# Autodesk Inventor assembly: 22205/20 E
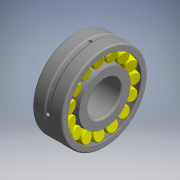
[picture p0: Inventor's stored thumbnail of the model, 180x180]
Saved by Autodesk Inventor 2017.3 (Build 213256000, 256)
## iProperties
Category: PARTsolutions
Company: SKF
Part Number: 22205/20 E
Catalog Web Link: www.cadenas.de
Description: BS2_001-Spherical roller bearings
Vendor: SKF
Document SubType Name: Assembly
Designer: partserver
Manufacturer: SKF
Mass: 280 g
Surface Area: 167.54 cm^2
Volume: 24.1426 cm^3
Density: 11.5977 g/cm^3
Title: 22205/20 E
Author: Cadenas PARTsolutions
Comments: Spherical roller bearings
PSOL_IDENT_0: {$CADENAS_DATA\23d-libs\skf\bearings_units_and_housings\roller_bearings\spherical_roller_bearings\bs
PSOL_IDENT_1: 2_001.prj},179 {VTYP=3D},{STYP=ASSTAB},{NB=22205/20 E},{LINA=22205/20 E},{NN=BS2_001},{DATE=23.12.20
PSOL_IDENT_2: 20 07:01:43},{GEOMDATE=14.12.2020 11:44:40},{VERSION=},{LINEID=460970},{WBVAR=},{WBNUMERIC=}  {NB=22
PSOL_IDENT_3: 205/20 E},{LINA=22205/20 E},{KT=DUMMY},{DESIGNATION=22205/20 E},{VARIANT=CE1W33},{DESIGNX=Cylindrica
PSOL_IDENT_4: l bore},{SEAL=No seals},{SALG=NO},{BORE=20.000},{DD=20.000},{DD1=MIN},{D=52.000},{B=18.000},{DD2=31.
PSOL_IDENT_5: 300},{DD3=MIN},{D1=44.200},{B1=MIN},{B2=MIN},{B4=MIN},{B5=MIN},{BB=3.700},{K=2.000},{R12=1.000},{G=}
PSOL_IDENT_6: ,{G1=MIN},{TB=MIN},{ALPHA=12.8333},{R34=MIN},{PITCH=39.459},{DW=7.130},{LW=6.600},{DDAMIN=25.600},{D
PSOL_IDENT_7: DAMAX=MIN},{DBMIN=MIN},{DAMAX=46.400},{BAMIN=MIN},{RAMAX=1.000},{LOAD1=49.900},{LOAD2=44.000},{LOAD3=
PSOL_IDENT_8: 4.750},{SPEED1=13000},{SPEED2=17000},{PRA=},{PLA=},{Z=15.000},{II=2.000},{MASS=0.280},{MASS2=MIN},{S
PSOL_IDENT_9: LEEVE=},{POPULAR=},{BEARING=22205/20 E},{PPATH=parts/bs2_001_asmtpl.prj},{RAMAXX=1},{EE=0.35},{Y0=1.
PSOL_IDENT_10: 8},{R12X=1},{Y2=2.9},{ALPHAX=12.83333},{Y1=1.9},{DD1X=},{B1X=},{SLEEVEX=},{ALPHAXX=},{B2X=},{SUPRESS
PSOL_IDENT_11: ED=},{BBALG=3.700},{KALG=2.000}
NB: 22205/20 E
NN: BS2_001
NT: Spherical roller bearings
NBSYN: $DESIGNATION.
LINA: 22205/20 E
CATALOG: SKF
DESIGNATION: 22205/20 E
DESIGNX: Cylindrical bore
SEAL: No seals
BORE: 20
D: 52
B: 18
LOAD1: 49.9
LOAD2: 44
LOAD3: 4.75
SPEED1: 13000
SPEED2: 17000
SUPPLIER: SKF
ARTICLENO: 22205/20 E
BOMINFO: 22205/20 E
CREATOR: CADENAS GmbH
## Documents named in this file (6)
- e:\temp\worker_18\temp\exporttempdir_6528_6_YBdq6\format_0\22205_20 E.iam
- e:\temp\worker_18\temp\exporttempdir_6528_6_YBdq6\format_0\22205_20 E_dummy.ipt
- e:\temp\worker_18\temp\exporttempdir_6528_6_YBdq6\format_0\22205_20 E_ir.ipt
- e:\temp\worker_18\temp\exporttempdir_6528_6_YBdq6\format_0\22205_20 E_or.ipt
- e:\temp\worker_18\temp\exporttempdir_6528_6_YBdq6\format_0\22205_20 E_r1.ipt
- e:\temp\worker_18\temp\exporttempdir_6528_6_YBdq6\format_0\22205_20 E_r2.ipt
## Components (33 placed, 5 different names)
1. 22205_20 E_dummy:1 — dummy_XY@1 <-> ir_XY@2, dummy_Z@1 <-> ir_Z@2, dummy_YZ@1 <-> ir_YZ@2, dummy_XY@1 <-> or_XY@3, dummy_Z@1 <-> or_Z@3, dummy_YZ@1 <-> or_YZ@3, roller1_XY@1 <-> roller1_XY@4, roller1_Z@1 <-> roller1_Z@4, roller1_YZ@1 <-> roller1_YZ@4, roller1_XY@1 <-> roller2_XY@5, roller1_Z@1 <-> roller2_Z@5, roller1_YZ@1 <-> roller2_YZ@5, roller2_XY@1 <-> roller1_XY@6, roller2_Z@1 <-> roller1_Z@6, roller2_YZ@1 <-> roller1_YZ@6, roller2_XY@1 <-> roller2_XY@7, roller2_Z@1 <-> roller2_Z@7, roller2_YZ@1 <-> roller2_YZ@7, roller3_XY@1 <-> roller1_XY@8, roller3_Z@1 <-> roller1_Z@8, roller3_YZ@1 <-> roller1_YZ@8, roller3_XY@1 <-> roller2_XY@9, roller3_Z@1 <-> roller2_Z@9, roller3_YZ@1 <-> roller2_YZ@9, roller4_XY@1 <-> roller1_XY@10, roller4_Z@1 <-> roller1_Z@10, roller4_YZ@1 <-> roller1_YZ@10, roller4_XY@1 <-> roller2_XY@11, roller4_Z@1 <-> roller2_Z@11, roller4_YZ@1 <-> roller2_YZ@11, roller5_XY@1 <-> roller1_XY@12, roller5_Z@1 <-> roller1_Z@12, roller5_YZ@1 <-> roller1_YZ@12, roller5_XY@1 <-> roller2_XY@13, roller5_Z@1 <-> roller2_Z@13, roller5_YZ@1 <-> roller2_YZ@13, roller6_XY@1 <-> roller1_XY@14, roller6_Z@1 <-> roller1_Z@14, roller6_YZ@1 <-> roller1_YZ@14, roller6_XY@1 <-> roller2_XY@15, roller6_Z@1 <-> roller2_Z@15, roller6_YZ@1 <-> roller2_YZ@15, roller7_XY@1 <-> roller1_XY@16, roller7_Z@1 <-> roller1_Z@16, roller7_YZ@1 <-> roller1_YZ@16, roller7_XY@1 <-> roller2_XY@17, roller7_Z@1 <-> roller2_Z@17, roller7_YZ@1 <-> roller2_YZ@17, roller8_XY@1 <-> roller1_XY@18, roller8_Z@1 <-> roller1_Z@18, roller8_YZ@1 <-> roller1_YZ@18, roller8_XY@1 <-> roller2_XY@19, roller8_Z@1 <-> roller2_Z@19, roller8_YZ@1 <-> roller2_YZ@19, roller9_XY@1 <-> roller1_XY@20, roller9_Z@1 <-> roller1_Z@20, roller9_YZ@1 <-> roller1_YZ@20, roller9_XY@1 <-> roller2_XY@21, roller9_Z@1 <-> roller2_Z@21, roller9_YZ@1 <-> roller2_YZ@21, roller10_XY@1 <-> roller1_XY@22, roller10_Z@1 <-> roller1_Z@22, roller10_YZ@1 <-> roller1_YZ@22, roller10_XY@1 <-> roller2_XY@23, roller10_Z@1 <-> roller2_Z@23, roller10_YZ@1 <-> roller2_YZ@23, roller11_XY@1 <-> roller1_XY@24, roller11_Z@1 <-> roller1_Z@24, roller11_YZ@1 <-> roller1_YZ@24, roller11_XY@1 <-> roller2_XY@25, roller11_Z@1 <-> roller2_Z@25, roller11_YZ@1 <-> roller2_YZ@25, roller12_XY@1 <-> roller1_XY@26, roller12_Z@1 <-> roller1_Z@26, roller12_YZ@1 <-> roller1_YZ@26, roller12_XY@1 <-> roller2_XY@27, roller12_Z@1 <-> roller2_Z@27, roller12_YZ@1 <-> roller2_YZ@27, roller13_XY@1 <-> roller1_XY@28, roller13_Z@1 <-> roller1_Z@28, roller13_YZ@1 <-> roller1_YZ@28, roller13_XY@1 <-> roller2_XY@29, roller13_Z@1 <-> roller2_Z@29, roller13_YZ@1 <-> roller2_YZ@29, roller14_XY@1 <-> roller1_XY@30, roller14_Z@1 <-> roller1_Z@30, roller14_YZ@1 <-> roller1_YZ@30, roller14_XY@1 <-> roller2_XY@31, roller14_Z@1 <-> roller2_Z@31, roller14_YZ@1 <-> roller2_YZ@31, roller15_XY@1 <-> roller1_XY@32, roller15_Z@1 <-> roller1_Z@32, roller15_YZ@1 <-> roller1_YZ@32, roller15_XY@1 <-> roller2_XY@33, roller15_Z@1 <-> roller2_Z@33, roller15_YZ@1 <-> roller2_YZ@33
2. 22205_20 E_ir:1 — dummy_XY@1 <-> ir_XY@2, dummy_Z@1 <-> ir_Z@2, dummy_YZ@1 <-> ir_YZ@2
3. 22205_20 E_or:1 — dummy_XY@1 <-> or_XY@3, dummy_Z@1 <-> or_Z@3, dummy_YZ@1 <-> or_YZ@3
4. 22205_20 E_r1:1 — roller1_XY@1 <-> roller1_XY@4, roller1_Z@1 <-> roller1_Z@4, roller1_YZ@1 <-> roller1_YZ@4
5. 22205_20 E_r2:1 — roller1_XY@1 <-> roller2_XY@5, roller1_Z@1 <-> roller2_Z@5, roller1_YZ@1 <-> roller2_YZ@5
6. 22205_20 E_r1:2 — roller2_XY@1 <-> roller1_XY@6, roller2_Z@1 <-> roller1_Z@6, roller2_YZ@1 <-> roller1_YZ@6
7. 22205_20 E_r2:2 — roller2_XY@1 <-> roller2_XY@7, roller2_Z@1 <-> roller2_Z@7, roller2_YZ@1 <-> roller2_YZ@7
8. 22205_20 E_r1:3 — roller3_XY@1 <-> roller1_XY@8, roller3_Z@1 <-> roller1_Z@8, roller3_YZ@1 <-> roller1_YZ@8
9. 22205_20 E_r2:3 — roller3_XY@1 <-> roller2_XY@9, roller3_Z@1 <-> roller2_Z@9, roller3_YZ@1 <-> roller2_YZ@9
10. 22205_20 E_r1:4 — roller4_XY@1 <-> roller1_XY@10, roller4_Z@1 <-> roller1_Z@10, roller4_YZ@1 <-> roller1_YZ@10
11. 22205_20 E_r2:4 — roller4_XY@1 <-> roller2_XY@11, roller4_Z@1 <-> roller2_Z@11, roller4_YZ@1 <-> roller2_YZ@11
12. 22205_20 E_r1:5 — roller5_XY@1 <-> roller1_XY@12, roller5_Z@1 <-> roller1_Z@12, roller5_YZ@1 <-> roller1_YZ@12
13. 22205_20 E_r2:5 — roller5_XY@1 <-> roller2_XY@13, roller5_Z@1 <-> roller2_Z@13, roller5_YZ@1 <-> roller2_YZ@13
14. 22205_20 E_r1:6 — roller6_XY@1 <-> roller1_XY@14, roller6_Z@1 <-> roller1_Z@14, roller6_YZ@1 <-> roller1_YZ@14
15. 22205_20 E_r2:6 — roller6_XY@1 <-> roller2_XY@15, roller6_Z@1 <-> roller2_Z@15, roller6_YZ@1 <-> roller2_YZ@15
16. 22205_20 E_r1:7 — roller7_XY@1 <-> roller1_XY@16, roller7_Z@1 <-> roller1_Z@16, roller7_YZ@1 <-> roller1_YZ@16
17. 22205_20 E_r2:7 — roller7_XY@1 <-> roller2_XY@17, roller7_Z@1 <-> roller2_Z@17, roller7_YZ@1 <-> roller2_YZ@17
18. 22205_20 E_r1:8 — roller8_XY@1 <-> roller1_XY@18, roller8_Z@1 <-> roller1_Z@18, roller8_YZ@1 <-> roller1_YZ@18
19. 22205_20 E_r2:8 — roller8_XY@1 <-> roller2_XY@19, roller8_Z@1 <-> roller2_Z@19, roller8_YZ@1 <-> roller2_YZ@19
20. 22205_20 E_r1:9 — roller9_XY@1 <-> roller1_XY@20, roller9_Z@1 <-> roller1_Z@20, roller9_YZ@1 <-> roller1_YZ@20
21. 22205_20 E_r2:9 — roller9_XY@1 <-> roller2_XY@21, roller9_Z@1 <-> roller2_Z@21, roller9_YZ@1 <-> roller2_YZ@21
22. 22205_20 E_r1:10 — roller10_XY@1 <-> roller1_XY@22, roller10_Z@1 <-> roller1_Z@22, roller10_YZ@1 <-> roller1_YZ@22
23. 22205_20 E_r2:10 — roller10_XY@1 <-> roller2_XY@23, roller10_Z@1 <-> roller2_Z@23, roller10_YZ@1 <-> roller2_YZ@23
24. 22205_20 E_r1:11 — roller11_XY@1 <-> roller1_XY@24, roller11_Z@1 <-> roller1_Z@24, roller11_YZ@1 <-> roller1_YZ@24
25. 22205_20 E_r2:11 — roller11_XY@1 <-> roller2_XY@25, roller11_Z@1 <-> roller2_Z@25, roller11_YZ@1 <-> roller2_YZ@25
26. 22205_20 E_r1:12 — roller12_XY@1 <-> roller1_XY@26, roller12_Z@1 <-> roller1_Z@26, roller12_YZ@1 <-> roller1_YZ@26
27. 22205_20 E_r2:12 — roller12_XY@1 <-> roller2_XY@27, roller12_Z@1 <-> roller2_Z@27, roller12_YZ@1 <-> roller2_YZ@27
28. 22205_20 E_r1:13 — roller13_XY@1 <-> roller1_XY@28, roller13_Z@1 <-> roller1_Z@28, roller13_YZ@1 <-> roller1_YZ@28
29. 22205_20 E_r2:13 — roller13_XY@1 <-> roller2_XY@29, roller13_Z@1 <-> roller2_Z@29, roller13_YZ@1 <-> roller2_YZ@29
30. 22205_20 E_r1:14 — roller14_XY@1 <-> roller1_XY@30, roller14_Z@1 <-> roller1_Z@30, roller14_YZ@1 <-> roller1_YZ@30
31. 22205_20 E_r2:14 — roller14_XY@1 <-> roller2_XY@31, roller14_Z@1 <-> roller2_Z@31, roller14_YZ@1 <-> roller2_YZ@31
32. 22205_20 E_r1:15 — roller15_XY@1 <-> roller1_XY@32, roller15_Z@1 <-> roller1_Z@32, roller15_YZ@1 <-> roller1_YZ@32
33. 22205_20 E_r2:15 — roller15_XY@1 <-> roller2_XY@33, roller15_Z@1 <-> roller2_Z@33, roller15_YZ@1 <-> roller2_YZ@33
## Relationships (96: Mate 34, Angle 32, Flush 30)
- dummy_XY@1 <-> ir_XY@2 [Mate]: 22205_20 E_dummy:1 ↔ 22205_20 E_ir:1
- dummy_Z@1 <-> ir_Z@2 [Mate]: 22205_20 E_dummy:1 ↔ 22205_20 E_ir:1
- dummy_YZ@1 <-> ir_YZ@2 [Angle] (0 deg): 22205_20 E_dummy:1 ↔ 22205_20 E_ir:1
- dummy_XY@1 <-> or_XY@3 [Mate]: 22205_20 E_dummy:1 ↔ 22205_20 E_or:1
- dummy_Z@1 <-> or_Z@3 [Mate]: 22205_20 E_dummy:1 ↔ 22205_20 E_or:1
- dummy_YZ@1 <-> or_YZ@3 [Angle] (0 deg): 22205_20 E_dummy:1 ↔ 22205_20 E_or:1
- roller1_XY@1 <-> roller1_XY@4 [Flush]: 22205_20 E_dummy:1 ↔ 22205_20 E_r1:1
- roller1_Z@1 <-> roller1_Z@4 [Mate]: 22205_20 E_dummy:1 ↔ 22205_20 E_r1:1
- roller1_YZ@1 <-> roller1_YZ@4 [Angle] (0 deg): 22205_20 E_dummy:1 ↔ 22205_20 E_r1:1
- roller1_XY@1 <-> roller2_XY@5 [Flush]: 22205_20 E_dummy:1 ↔ 22205_20 E_r2:1
- roller1_Z@1 <-> roller2_Z@5 [Mate]: 22205_20 E_dummy:1 ↔ 22205_20 E_r2:1
- roller1_YZ@1 <-> roller2_YZ@5 [Angle] (0 deg): 22205_20 E_dummy:1 ↔ 22205_20 E_r2:1
- roller2_XY@1 <-> roller1_XY@6 [Flush]: 22205_20 E_dummy:1 ↔ 22205_20 E_r1:2
- roller2_Z@1 <-> roller1_Z@6 [Mate]: 22205_20 E_dummy:1 ↔ 22205_20 E_r1:2
- roller2_YZ@1 <-> roller1_YZ@6 [Angle] (0 deg): 22205_20 E_dummy:1 ↔ 22205_20 E_r1:2
- roller2_XY@1 <-> roller2_XY@7 [Flush]: 22205_20 E_dummy:1 ↔ 22205_20 E_r2:2
- roller2_Z@1 <-> roller2_Z@7 [Mate]: 22205_20 E_dummy:1 ↔ 22205_20 E_r2:2
- roller2_YZ@1 <-> roller2_YZ@7 [Angle] (0 deg): 22205_20 E_dummy:1 ↔ 22205_20 E_r2:2
- roller3_XY@1 <-> roller1_XY@8 [Flush]: 22205_20 E_dummy:1 ↔ 22205_20 E_r1:3
- roller3_Z@1 <-> roller1_Z@8 [Mate]: 22205_20 E_dummy:1 ↔ 22205_20 E_r1:3
- roller3_YZ@1 <-> roller1_YZ@8 [Angle] (0 deg): 22205_20 E_dummy:1 ↔ 22205_20 E_r1:3
- roller3_XY@1 <-> roller2_XY@9 [Flush]: 22205_20 E_dummy:1 ↔ 22205_20 E_r2:3
- roller3_Z@1 <-> roller2_Z@9 [Mate]: 22205_20 E_dummy:1 ↔ 22205_20 E_r2:3
- roller3_YZ@1 <-> roller2_YZ@9 [Angle] (0 deg): 22205_20 E_dummy:1 ↔ 22205_20 E_r2:3
- roller4_XY@1 <-> roller1_XY@10 [Flush]: 22205_20 E_dummy:1 ↔ 22205_20 E_r1:4
- roller4_Z@1 <-> roller1_Z@10 [Mate]: 22205_20 E_dummy:1 ↔ 22205_20 E_r1:4
- roller4_YZ@1 <-> roller1_YZ@10 [Angle] (0 deg): 22205_20 E_dummy:1 ↔ 22205_20 E_r1:4
- roller4_XY@1 <-> roller2_XY@11 [Flush]: 22205_20 E_dummy:1 ↔ 22205_20 E_r2:4
- roller4_Z@1 <-> roller2_Z@11 [Mate]: 22205_20 E_dummy:1 ↔ 22205_20 E_r2:4
- roller4_YZ@1 <-> roller2_YZ@11 [Angle] (0 deg): 22205_20 E_dummy:1 ↔ 22205_20 E_r2:4
- roller5_XY@1 <-> roller1_XY@12 [Flush]: 22205_20 E_dummy:1 ↔ 22205_20 E_r1:5
- roller5_Z@1 <-> roller1_Z@12 [Mate]: 22205_20 E_dummy:1 ↔ 22205_20 E_r1:5
- roller5_YZ@1 <-> roller1_YZ@12 [Angle] (0 deg): 22205_20 E_dummy:1 ↔ 22205_20 E_r1:5
- roller5_XY@1 <-> roller2_XY@13 [Flush]: 22205_20 E_dummy:1 ↔ 22205_20 E_r2:5
- roller5_Z@1 <-> roller2_Z@13 [Mate]: 22205_20 E_dummy:1 ↔ 22205_20 E_r2:5
- roller5_YZ@1 <-> roller2_YZ@13 [Angle] (0 deg): 22205_20 E_dummy:1 ↔ 22205_20 E_r2:5
- roller6_XY@1 <-> roller1_XY@14 [Flush]: 22205_20 E_dummy:1 ↔ 22205_20 E_r1:6
- roller6_Z@1 <-> roller1_Z@14 [Mate]: 22205_20 E_dummy:1 ↔ 22205_20 E_r1:6
- roller6_YZ@1 <-> roller1_YZ@14 [Angle] (0 deg): 22205_20 E_dummy:1 ↔ 22205_20 E_r1:6
- roller6_XY@1 <-> roller2_XY@15 [Flush]: 22205_20 E_dummy:1 ↔ 22205_20 E_r2:6
- roller6_Z@1 <-> roller2_Z@15 [Mate]: 22205_20 E_dummy:1 ↔ 22205_20 E_r2:6
- roller6_YZ@1 <-> roller2_YZ@15 [Angle] (0 deg): 22205_20 E_dummy:1 ↔ 22205_20 E_r2:6
- roller7_XY@1 <-> roller1_XY@16 [Flush]: 22205_20 E_dummy:1 ↔ 22205_20 E_r1:7
- roller7_Z@1 <-> roller1_Z@16 [Mate]: 22205_20 E_dummy:1 ↔ 22205_20 E_r1:7
- roller7_YZ@1 <-> roller1_YZ@16 [Angle] (0 deg): 22205_20 E_dummy:1 ↔ 22205_20 E_r1:7
- roller7_XY@1 <-> roller2_XY@17 [Flush]: 22205_20 E_dummy:1 ↔ 22205_20 E_r2:7
- roller7_Z@1 <-> roller2_Z@17 [Mate]: 22205_20 E_dummy:1 ↔ 22205_20 E_r2:7
- roller7_YZ@1 <-> roller2_YZ@17 [Angle] (0 deg): 22205_20 E_dummy:1 ↔ 22205_20 E_r2:7
- roller8_XY@1 <-> roller1_XY@18 [Flush]: 22205_20 E_dummy:1 ↔ 22205_20 E_r1:8
- roller8_Z@1 <-> roller1_Z@18 [Mate]: 22205_20 E_dummy:1 ↔ 22205_20 E_r1:8
- roller8_YZ@1 <-> roller1_YZ@18 [Angle] (0 deg): 22205_20 E_dummy:1 ↔ 22205_20 E_r1:8
- roller8_XY@1 <-> roller2_XY@19 [Flush]: 22205_20 E_dummy:1 ↔ 22205_20 E_r2:8
- roller8_Z@1 <-> roller2_Z@19 [Mate]: 22205_20 E_dummy:1 ↔ 22205_20 E_r2:8
- roller8_YZ@1 <-> roller2_YZ@19 [Angle] (0 deg): 22205_20 E_dummy:1 ↔ 22205_20 E_r2:8
- roller9_XY@1 <-> roller1_XY@20 [Flush]: 22205_20 E_dummy:1 ↔ 22205_20 E_r1:9
- roller9_Z@1 <-> roller1_Z@20 [Mate]: 22205_20 E_dummy:1 ↔ 22205_20 E_r1:9
- roller9_YZ@1 <-> roller1_YZ@20 [Angle] (0 deg): 22205_20 E_dummy:1 ↔ 22205_20 E_r1:9
- roller9_XY@1 <-> roller2_XY@21 [Flush]: 22205_20 E_dummy:1 ↔ 22205_20 E_r2:9
- roller9_Z@1 <-> roller2_Z@21 [Mate]: 22205_20 E_dummy:1 ↔ 22205_20 E_r2:9
- roller9_YZ@1 <-> roller2_YZ@21 [Angle] (0 deg): 22205_20 E_dummy:1 ↔ 22205_20 E_r2:9
- roller10_XY@1 <-> roller1_XY@22 [Flush]: 22205_20 E_dummy:1 ↔ 22205_20 E_r1:10
- roller10_Z@1 <-> roller1_Z@22 [Mate]: 22205_20 E_dummy:1 ↔ 22205_20 E_r1:10
- roller10_YZ@1 <-> roller1_YZ@22 [Angle] (0 deg): 22205_20 E_dummy:1 ↔ 22205_20 E_r1:10
- roller10_XY@1 <-> roller2_XY@23 [Flush]: 22205_20 E_dummy:1 ↔ 22205_20 E_r2:10
- roller10_Z@1 <-> roller2_Z@23 [Mate]: 22205_20 E_dummy:1 ↔ 22205_20 E_r2:10
- roller10_YZ@1 <-> roller2_YZ@23 [Angle] (0 deg): 22205_20 E_dummy:1 ↔ 22205_20 E_r2:10
- roller11_XY@1 <-> roller1_XY@24 [Flush]: 22205_20 E_dummy:1 ↔ 22205_20 E_r1:11
- roller11_Z@1 <-> roller1_Z@24 [Mate]: 22205_20 E_dummy:1 ↔ 22205_20 E_r1:11
- roller11_YZ@1 <-> roller1_YZ@24 [Angle] (0 deg): 22205_20 E_dummy:1 ↔ 22205_20 E_r1:11
- roller11_XY@1 <-> roller2_XY@25 [Flush]: 22205_20 E_dummy:1 ↔ 22205_20 E_r2:11
- roller11_Z@1 <-> roller2_Z@25 [Mate]: 22205_20 E_dummy:1 ↔ 22205_20 E_r2:11
- roller11_YZ@1 <-> roller2_YZ@25 [Angle] (0 deg): 22205_20 E_dummy:1 ↔ 22205_20 E_r2:11
- roller12_XY@1 <-> roller1_XY@26 [Flush]: 22205_20 E_dummy:1 ↔ 22205_20 E_r1:12
- roller12_Z@1 <-> roller1_Z@26 [Mate]: 22205_20 E_dummy:1 ↔ 22205_20 E_r1:12
- roller12_YZ@1 <-> roller1_YZ@26 [Angle] (0 deg): 22205_20 E_dummy:1 ↔ 22205_20 E_r1:12
- roller12_XY@1 <-> roller2_XY@27 [Flush]: 22205_20 E_dummy:1 ↔ 22205_20 E_r2:12
- roller12_Z@1 <-> roller2_Z@27 [Mate]: 22205_20 E_dummy:1 ↔ 22205_20 E_r2:12
- roller12_YZ@1 <-> roller2_YZ@27 [Angle] (0 deg): 22205_20 E_dummy:1 ↔ 22205_20 E_r2:12
- roller13_XY@1 <-> roller1_XY@28 [Flush]: 22205_20 E_dummy:1 ↔ 22205_20 E_r1:13
- roller13_Z@1 <-> roller1_Z@28 [Mate]: 22205_20 E_dummy:1 ↔ 22205_20 E_r1:13
- roller13_YZ@1 <-> roller1_YZ@28 [Angle] (0 deg): 22205_20 E_dummy:1 ↔ 22205_20 E_r1:13
- roller13_XY@1 <-> roller2_XY@29 [Flush]: 22205_20 E_dummy:1 ↔ 22205_20 E_r2:13
- roller13_Z@1 <-> roller2_Z@29 [Mate]: 22205_20 E_dummy:1 ↔ 22205_20 E_r2:13
- roller13_YZ@1 <-> roller2_YZ@29 [Angle] (0 deg): 22205_20 E_dummy:1 ↔ 22205_20 E_r2:13
- roller14_XY@1 <-> roller1_XY@30 [Flush]: 22205_20 E_dummy:1 ↔ 22205_20 E_r1:14
- roller14_Z@1 <-> roller1_Z@30 [Mate]: 22205_20 E_dummy:1 ↔ 22205_20 E_r1:14
- roller14_YZ@1 <-> roller1_YZ@30 [Angle] (0 deg): 22205_20 E_dummy:1 ↔ 22205_20 E_r1:14
- roller14_XY@1 <-> roller2_XY@31 [Flush]: 22205_20 E_dummy:1 ↔ 22205_20 E_r2:14
- roller14_Z@1 <-> roller2_Z@31 [Mate]: 22205_20 E_dummy:1 ↔ 22205_20 E_r2:14
- roller14_YZ@1 <-> roller2_YZ@31 [Angle] (0 deg): 22205_20 E_dummy:1 ↔ 22205_20 E_r2:14
- roller15_XY@1 <-> roller1_XY@32 [Flush]: 22205_20 E_dummy:1 ↔ 22205_20 E_r1:15
- roller15_Z@1 <-> roller1_Z@32 [Mate]: 22205_20 E_dummy:1 ↔ 22205_20 E_r1:15
- roller15_YZ@1 <-> roller1_YZ@32 [Angle] (0 deg): 22205_20 E_dummy:1 ↔ 22205_20 E_r1:15
- roller15_XY@1 <-> roller2_XY@33 [Flush]: 22205_20 E_dummy:1 ↔ 22205_20 E_r2:15
- roller15_Z@1 <-> roller2_Z@33 [Mate]: 22205_20 E_dummy:1 ↔ 22205_20 E_r2:15
- roller15_YZ@1 <-> roller2_YZ@33 [Angle] (0 deg): 22205_20 E_dummy:1 ↔ 22205_20 E_r2:15
